# Autodesk Inventor assembly: LinearActuator
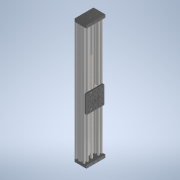
[picture p0: Inventor's stored thumbnail of the model, 180x180]
Saved by Autodesk Inventor 2022 (Build 260153000, 153)
## iProperties
Created: 2021-11-09
Part Number: LinearActuator
Document SubType Name: Assembly
Designer: JK
Author: JK
## Documents named in this file (11)
- C:\Users\JK\Documents\Inventor\UTM\LinearActuator.iam
- C:\Users\JK\Documents\Inventor\UTM\VSlotAluminiumProfile40x80x500mm.ipt
- C:\Users\JK\Documents\Inventor\UTM\BearingPlate.ipt
- C:\Users\JK\Documents\Inventor\UTM\SmallGantryCProfile.ipt
- C:\Users\JK\Documents\Inventor\UTM\EccentricSpacer.ipt
- C:\Users\JK\Documents\Inventor\UTM\AntiBacklashNut.ipt
- C:\Users\JK\Documents\Inventor\UTM\3mmSpacer.ipt
- C:\Users\JK\Documents\Inventor\UTM\6mmSpacer.ipt
- C:\Users\JK\Documents\Inventor\UTM\MiniWasher.ipt
- C:\Users\JK\Documents\Inventor\UTM\SmallWheel.ipt
- C:\Users\JK\Documents\Inventor\UTM\Trapezoidal lead screw tr8x8-4.ipt
## Components (20 placed, 10 different names)
1. VSlotAluminiumProfile40x80x500mm:1
2. BearingPlate:1
3. BearingPlate:2
4. SmallGantryCProfile:1
5. EccentricSpacer:1
6. EccentricSpacer:2
7. AntiBacklashNut:1 — Coincidencia:27
8. 3mmSpacer:1
9. 3mmSpacer:2
10. 6mmSpacer:1
11. 6mmSpacer:2
12. MiniWasher:1
13. MiniWasher:2
14. MiniWasher:3
15. MiniWasher:4
16. SmallWheel:1
17. SmallWheel:2
18. SmallWheel:3
19. SmallWheel:4
20. Trapezoidal lead screw tr8x8-4:1 — Coincidencia:27
## Relationships (39: Mate 27, Flush 11, Angle 1)
- [Mate]: VSlotAluminiumProfile40x80x500mm:1 ↔ BearingPlate:1
- [Mate]: VSlotAluminiumProfile40x80x500mm:1 ↔ BearingPlate:1
- [Flush]: VSlotAluminiumProfile40x80x500mm:1 ↔ BearingPlate:1
- [Mate]: VSlotAluminiumProfile40x80x500mm:1 ↔ BearingPlate:2
- [Mate]: BearingPlate:1 ↔ BearingPlate:2
- [Flush]: VSlotAluminiumProfile40x80x500mm:1 ↔ BearingPlate:2
- [Mate]: SmallGantryCProfile:1 ↔ AntiBacklashNut:1
- [Mate]: SmallGantryCProfile:1 ↔ AntiBacklashNut:1
- [Mate]: AntiBacklashNut:1 ↔ 3mmSpacer:1
- [Mate]: AntiBacklashNut:1 ↔ 3mmSpacer:2
- [Flush]: 3mmSpacer:1 ↔ 3mmSpacer:2
- [Mate]: AntiBacklashNut:1 ↔ 3mmSpacer:1
- [Mate]: SmallGantryCProfile:1 ↔ 3mmSpacer:1
- [Mate]: SmallGantryCProfile:1 ↔ EccentricSpacer:2
- [Mate]: SmallGantryCProfile:1 ↔ EccentricSpacer:1
- [Flush]: EccentricSpacer:1 ↔ EccentricSpacer:2
- [Mate]: SmallGantryCProfile:1 ↔ EccentricSpacer:2
- [Mate]: SmallGantryCProfile:1 ↔ 6mmSpacer:2
- [Mate]: SmallGantryCProfile:1 ↔ 6mmSpacer:1
- [Flush]: 6mmSpacer:1 ↔ 6mmSpacer:2
- [Mate]: SmallGantryCProfile:1 ↔ 6mmSpacer:2
- [Mate]: 6mmSpacer:2 ↔ MiniWasher:1
- [Mate]: EccentricSpacer:1 ↔ MiniWasher:2
- [Mate]: 6mmSpacer:1 ↔ MiniWasher:4
- [Mate]: EccentricSpacer:2 ↔ MiniWasher:3
- [Flush]: MiniWasher:1 ↔ MiniWasher:2
- [Flush]: MiniWasher:1 ↔ MiniWasher:4
- [Flush]: MiniWasher:2 ↔ MiniWasher:3
- [Mate]: EccentricSpacer:1 ↔ MiniWasher:2
- [Flush]: SmallWheel:3 ↔ SmallWheel:4
- [Flush]: SmallWheel:1 ↔ SmallWheel:3
- [Flush]: SmallWheel:1 ↔ SmallWheel:2
- [Mate]: 6mmSpacer:2 ↔ SmallWheel:1
- [Mate]: EccentricSpacer:1 ↔ SmallWheel:3
- [Mate]: MiniWasher:3 ↔ SmallWheel:2
- [Mate]: 6mmSpacer:1 ↔ SmallWheel:4
- [Mate]: MiniWasher:2 ↔ SmallWheel:3
- [Angle] (180 deg): BearingPlate:2 ↔ SmallGantryCProfile:1
- Coincidencia:27 [Mate]: AntiBacklashNut:1 ↔ Trapezoidal lead screw tr8x8-4:1
## Named parameters: d1_d11 = 0 mm, d2_d12 = 0 mm, d3_d13 = 0 mm, d4_d14 = 0 mm, d5_d15 = 0 mm, d6_d16 = 0 mm, d7_d17 = 0 mm, d8_d18 = 0 mm, d9_d19 = 0 mm, d10_d20 = 0 mm, d11_d21 = 0 mm, d12_d22 = 0 mm, d13_d23 = 0 mm, d14_d24 = 0 mm, d15_d25 = 0 mm, d16_d26 = 0 mm, d17_d27 = 0 mm, d18_d28 = 0 mm, d19_d29 = 0 mm, d20_d30 = 0 mm, d21_d31 = 0 mm, d22_d32 = 0 mm, d23_d33 = 0 mm, d24_d36 = 0 mm, d25_d37 = 0 mm
